# Autodesk Inventor assembly: 5 Barras Version 0
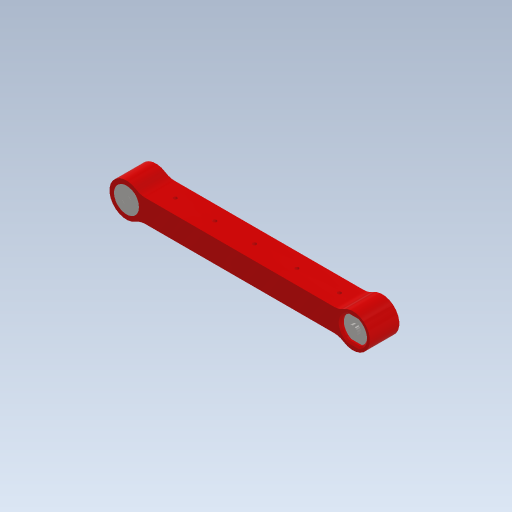
[picture p0: Inventor's stored thumbnail of the model, 512x512]
Saved by Autodesk Inventor 2024.2 (Build 282272000, 272)
## iProperties
Created: 2025-02-06
Part Number: 5 Barras Version 0
Document SubType Name: Assembly
Designer: jp.reyesf
Mass: 262.653 g
Surface Area: 368.793 cm^2
Volume: 121.736 cm^3
Density: 2.15757 g/cm^3
Author: jp.reyesf
## Documents named in this file (7)
- C:\Users\jp.reyesf\Desktop\Master-Thesis\five_bar\assets\CAD\Robot\Subassemblies\Distal Link 1.iam
- C:\Users\jp.reyesf\Desktop\Master-Thesis\five_bar\assets\CAD\Robot\Distal Link 2.ipt
- C:\Users\jp.reyesf\Desktop\Master-Thesis\five_bar\assets\CAD\Robot\Spacer.ipt
- C:\Users\jp.reyesf\Desktop\Master-Thesis\five_bar\assets\CAD\Robot\Bearing.ipt
- C:\Users\jp.reyesf\Desktop\Master-Thesis\five_bar\assets\CAD\Robot\separator.ipt
- C:\Users\jp.reyesf\Desktop\Master-Thesis\five_bar\assets\CAD\Robot\rod.ipt
- C:\Users\jp.reyesf\Desktop\Master-Thesis\five_bar\assets\CAD\Robot\Subassemblies\DummyBar.ipt
## Components (11 placed, 6 different names)
1. Distal Link 2:1 — Mate:33, Mate:34, Flush:8, Mate:53, Mate:55, Angle:1, Flush:9, Mate:56, Mate:57, Mate:58, Flush:10, Flush:11, Flush:12, Flush:13
2. Spacer:1 — Mate:6, Mate:7, Mate:8, Mate:9, Mate:33
3. Bearing:1 — Mate:6, Mate:8
4. separator:3 — Mate:54, Mate:56
5. Bearing:3 — Mate:7, Mate:9, Flush:12
6. Spacer:3 — Mate:34
7. Bearing:6 — Flush:13
8. Bearing:7
9. rod:2 — Flush:8, Mate:53, Mate:54
10. DummyBar:1 — Mate:57, Flush:11
11. DummyBar:2 — Mate:58, Flush:10
## Relationships (23: Mate 16, Flush 6, Angle 1)
- Mate:6: Spacer:1 ↔ Bearing:1
- Mate:7: Spacer:1 ↔ Bearing:3
- Mate:8: Spacer:1 ↔ Bearing:1
- Mate:9: Spacer:1 ↔ Bearing:3
- [Mate]: Spacer:3 ↔ Bearing:6
- [Mate]: Spacer:3 ↔ Bearing:7
- [Mate]: Spacer:3 ↔ Bearing:6
- [Mate]: Spacer:3 ↔ Bearing:7
- Mate:33: Distal Link 2:1 ↔ Spacer:1
- Mate:34: Distal Link 2:1 ↔ Spacer:3
- Flush:8: Distal Link 2:1 ↔ rod:2
- Mate:53: Distal Link 2:1 ↔ rod:2
- Mate:54: separator:3 ↔ rod:2
- Mate:55: Distal Link 2:1
- Angle:1 (180 deg): Distal Link 2:1
- Flush:9: Distal Link 2:1
- Mate:56: Distal Link 2:1 ↔ separator:3
- Mate:57: Distal Link 2:1 ↔ DummyBar:1
- Mate:58: Distal Link 2:1 ↔ DummyBar:2
- Flush:10: Distal Link 2:1 ↔ DummyBar:2
- Flush:11: Distal Link 2:1 ↔ DummyBar:1
- Flush:12: Distal Link 2:1 ↔ Bearing:3
- Flush:13: Distal Link 2:1 ↔ Bearing:6
## Named parameters: d22_d14 = 0 mm, d23_d15 = 0 mm, d24_d16 = 0 mm, d25_d17 = 0 mm
